# Autodesk Inventor assembly: DIL28-Socket+Package-Wide
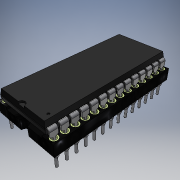
[picture p0: Inventor's stored thumbnail of the model, 180x180]
Saved by Autodesk Inventor 2018 (Build 220112000, 112)
## iProperties
Created: 2020-04-20
Part Number: DIL28-Socket+Package-Wide
Material: Všeobecné
Document SubType Name: Assembly
Designer: Jozko Mrkvicka
Author: Jozko Mrkvicka
## Documents named in this file (3)
- F:\Workspace\Projekty\Library\DIL28-Socket+Package-Wide.iam
- F:\Workspace\Projekty\Library\DIL28-Package-Wide.ipt
- F:\Workspace\Projekty\Library\DIL28-Socket-Wide.ipt
## Components (2 placed, 2 different names)
1. DIL28-Package-Wide:1 — Vložit:1, Proti sobě:1
2. DIL28-Socket-Wide:1 — Vložit:1, Proti sobě:1
## Relationships (2: Insert 1, Mate 1)
- Vložit:1 [Insert]: DIL28-Package-Wide:1 ↔ DIL28-Socket-Wide:1
- Proti sobě:1 [Mate]: DIL28-Package-Wide:1 ↔ DIL28-Socket-Wide:1
